# Autodesk Inventor assembly: [Midterm]CFD
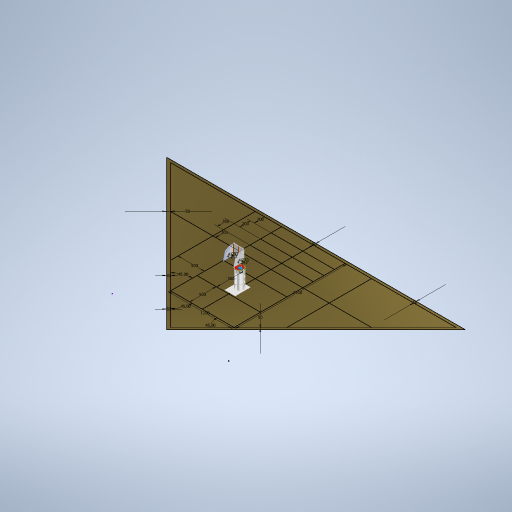
[picture p0: Inventor's stored thumbnail of the model, 512x512]
Saved by Autodesk Inventor 2024 (Build 280153000, 153)
## iProperties
Created: 2024-04-14
Part Number: [Midterm]CFD
Document SubType Name: Assembly
Designer: USER
Author: USER
## Documents named in this file (4)
- E:\university\大三\大三下\機工實務\圖檔\DesignVer2\[Midterm]CFD.iam
- E:\university\大三\大三下\機工實務\圖檔\DesignVer2\[Midterm]場地.ipt
- E:\university\大三\大三下\機工實務\圖檔\DesignVer2\[Midterm]Design.iam
- E:\university\大三\大三下\機工實務\圖檔\DesignVer2\[Midterm]場地(下部).ipt
## Components (3 placed, 3 different names)
1. [Midterm]場地:1 — 角度:1, 貼合:1, 齊平:1, 齊平:2
2. [Midterm]Design:1 [sub-assembly] — 角度:1, 貼合:2, 貼合:3
3. [Midterm]場地(下部):1 — 貼合:1, 齊平:1, 齊平:2, 貼合:2, 貼合:3
## Relationships (6: Mate 3, Flush 2, Angle 1)
- 角度:1 [Angle] (0 deg): [Midterm]場地:1 ↔ [Midterm]Design:1
- 貼合:1 [Mate]: [Midterm]場地:1 ↔ [Midterm]場地(下部):1
- 齊平:1 [Flush]: [Midterm]場地:1 ↔ [Midterm]場地(下部):1
- 齊平:2 [Flush]: [Midterm]場地:1 ↔ [Midterm]場地(下部):1
- 貼合:2 [Mate] (22.3 mm): [Midterm]Design:1 ↔ [Midterm]場地(下部):1
- 貼合:3 [Mate]: [Midterm]Design:1 ↔ [Midterm]場地(下部):1
